# Autodesk Inventor assembly: Hydraulic Assembly
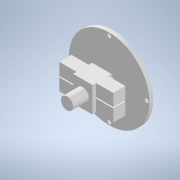
[picture p0: Inventor's stored thumbnail of the model, 180x180]
Saved by Autodesk Inventor 2021 (Build 250183000, 183)
## iProperties
Created: 2020-10-19
Part Number: Hydraulic Assembly
Document SubType Name: Assembly
Designer: jtri402
Author: jtri402
## Documents named in this file (3)
- D:\Uni y2\Sem2\236\Design Project\Assembly 4\assembly 4-20201020T195157Z-001\assembly 4\Hydraulic Assembly.iam
- D:\Uni y2\Sem2\236\Design Project\Assembly 4\assembly 4-20201020T195157Z-001\assembly 4\Rotary Motor Coupling.ipt
- D:\Uni y2\Sem2\236\Design Project\Assembly 4\assembly 4-20201020T195157Z-001\assembly 4\Semi Rotary Hydraulic Motor.ipt
## Components (2 placed, 2 different names)
1. Rotary Motor Coupling:1 — Rigid:1
2. Semi Rotary Hydraulic Motor:1 — Rigid:1
## Relationships (1: WeldJoint 1)
- Rigid:1 [WeldJoint]: Rotary Motor Coupling:1 ↔ Semi Rotary Hydraulic Motor:1
